# Autodesk Inventor assembly: КВ33.000.100 - Блок переключение передач
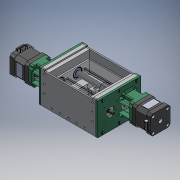
[picture p0: Inventor's stored thumbnail of the model, 180x180]
Saved by Autodesk Inventor 2019 (Build 230136000, 136)
## iProperties
Created: 2021-02-22
Part Number: КВ33.000.100 - Блок переключение передач
Material: Типовые
Document SubType Name: Assembly
Designer: Петров Иван
Author: Петров Иван
## Documents named in this file (13)
- E:\IVAN\Ivan_desktop\Kvantorium\Projects\tractor\design\КВ33.000.100 - Блок переключение передач.iam
- E:\IVAN\Ivan_desktop\Kvantorium\Projects\tractor\design\КВ33.000.101 - Площадка крепежная.ipt
- E:\IVAN\Ivan_desktop\Kvantorium\Projects\tractor\design\design_models\крышка КП.ipt
- E:\IVAN\Ivan_desktop\Kvantorium\Projects\tractor\design\КВ33.000.102 - Стенка толстая.ipt
- E:\IVAN\Ivan_desktop\Kvantorium\Projects\tractor\design\standart_components\Подшипник 626Z.ipt
- E:\IVAN\Ivan_desktop\Kvantorium\Projects\tractor\design\КВ33.000.103 - Стенка тонкая.ipt
- C:\Users\Петров Иван\Documents\Inventor\Content Center Files\R2019\en-US\AS 1427(03)\AS 1427 - M3,5 x 10(1).ipt
- E:\IVAN\Ivan_desktop\Kvantorium\Projects\tractor\design\КВ33.000.104 - Вал.ipt
- E:\IVAN\Ivan_desktop\Kvantorium\Projects\tractor\design\КВ33.000.105 - Каретка.ipt
- E:\IVAN\Ivan_desktop\Kvantorium\Projects\tractor\design\КВ33.000.106 - Муфта.ipt
- E:\IVAN\Ivan_desktop\Kvantorium\Projects\tractor\design\КВ33.000.107 - Крепеж мотора.ipt
- E:\IVAN\Ivan_desktop\Kvantorium\Projects\tractor\design\standart_components\nema 17 motor.ipt
- E:\IVAN\Ivan_desktop\Kvantorium\Projects\tractor\design\for manufacturing\step\КВ33.000.108 - Заслонка.ipt
## Components (43 placed, 12 different names)
1. крышка КП:1 — Flush:1, Mate:1, Mate:2
2. КВ33.000.101 - Площадка крепежная:1 — Flush:1, Mate:1, Mate:2, Mate:3, Flush:2, Mate:4, Mate:5, Flush:3, Mate:6
3. КВ33.000.102 - Стенка толстая:1 — Mate:5, Flush:3, Mate:6, Insert:3, Insert:4, Mate:13, Mate:14, Mate:15, Mate:16, Mate:17, Mate:23, Mate:26, Mate:27, Mate:29, Flush:5, Mate:32, Mate:37, Flush:6, Mate:58, Mate:61
4. КВ33.000.102 - Стенка толстая:2 — Mate:3, Flush:2, Mate:4, Insert:1, Insert:2, Flush:4, Mate:18, Mate:19, Mate:20, Mate:21, Mate:22, Mate:24, Mate:25, Mate:36, Flush:7, Mate:40, Mate:59, Mate:60
5. Подшипник 626Z:1 — Insert:1
6. Подшипник 626Z:2 — Insert:2
7. Подшипник 626Z:3 — Insert:3, Mate:28
8. Подшипник 626Z:4 — Insert:4
9. КВ33.000.103 - Стенка тонкая:1 — Flush:4, Mate:24, Mate:25, Mate:26
10. КВ33.000.103 - Стенка тонкая:2 — Mate:23, Mate:57
11. КВ33.000.104 - Вал:1 — Mate:27, Mate:28, Mate:30, Mate:55
12. КВ33.000.104 - Вал:2 — Mate:29, Flush:5, Mate:31, Mate:34, Mate:56
13. КВ33.000.105 - Каретка:1 — Mate:30, Tangent:1, Mate:60
14. КВ33.000.105 - Каретка:2 — Mate:31, Mate:61, Tangent:2
15. КВ33.000.106 - Муфта:1 — Mate:32, Mate:38, Mate:55
16. КВ33.000.106 - Муфта:2 — Mate:34, Mate:36, Mate:39, Mate:56
17. КВ33.000.107 - Крепеж мотора:1 — Mate:39, Flush:7, Mate:40, Mate:41, Flush:8, Flush:9, Mate:49, Mate:50, Mate:51, Mate:52, Mate:53, Mate:54
18. КВ33.000.107 - Крепеж мотора:2 — Mate:37, Mate:38, Flush:6, Flush:10, Flush:11, Mate:42, Mate:43, Mate:44, Mate:45, Mate:46, Mate:47, Mate:48
19. nema 17 motor:1 — Mate:41, Flush:8, Flush:9
20. nema 17 motor:2 — Flush:10, Flush:11, Mate:42
21. КВ33.000.108 - Заслонка:1 — Mate:57, Mate:58, Mate:59, Tangent:1, Tangent:2
22. AS 1427 - Metric M3,5 x 10:11 — Mate:43
23. AS 1427 - Metric M3,5 x 10:12 — Mate:44
24. AS 1427 - Metric M3,5 x 10:13 — Mate:45
25. AS 1427 - Metric M3,5 x 10:14 — Mate:46
26. AS 1427 - Metric M3,5 x 10:15 — Mate:47
27. AS 1427 - Metric M3,5 x 10:16 — Mate:48
28. AS 1427 - Metric M3,5 x 10:17 — Mate:49
29. AS 1427 - Metric M3,5 x 10:18 — Mate:50
30. AS 1427 - Metric M3,5 x 10:19 — Mate:51
31. AS 1427 - Metric M3,5 x 10:20 — Mate:52
32. AS 1427 - Metric M3,5 x 10:21 — Mate:53
33. AS 1427 - Metric M3,5 x 10:22 — Mate:54
34. AS 1427 - Metric M3,5 x 10:1 — Mate:13
35. AS 1427 - Metric M3,5 x 10:2 — Mate:14
36. AS 1427 - Metric M3,5 x 10:3 — Mate:15
37. AS 1427 - Metric M3,5 x 10:4 — Mate:16
38. AS 1427 - Metric M3,5 x 10:5 — Mate:17
39. AS 1427 - Metric M3,5 x 10:6 — Mate:18
40. AS 1427 - Metric M3,5 x 10:7 — Mate:19
41. AS 1427 - Metric M3,5 x 10:8 — Mate:20
42. AS 1427 - Metric M3,5 x 10:9 — Mate:21
43. AS 1427 - Metric M3,5 x 10:10 — Mate:22
## Relationships (70: Mate 53, Flush 11, Insert 4, Tangent 2)
- Flush:1 (-15 mm): крышка КП:1 ↔ КВ33.000.101 - Площадка крепежная:1
- Mate:1: крышка КП:1 ↔ КВ33.000.101 - Площадка крепежная:1
- Mate:2: крышка КП:1 ↔ КВ33.000.101 - Площадка крепежная:1
- Mate:3: КВ33.000.101 - Площадка крепежная:1 ↔ КВ33.000.102 - Стенка толстая:2
- Flush:2: КВ33.000.101 - Площадка крепежная:1 ↔ КВ33.000.102 - Стенка толстая:2
- Mate:4: КВ33.000.101 - Площадка крепежная:1 ↔ КВ33.000.102 - Стенка толстая:2
- Mate:5: КВ33.000.101 - Площадка крепежная:1 ↔ КВ33.000.102 - Стенка толстая:1
- Flush:3: КВ33.000.101 - Площадка крепежная:1 ↔ КВ33.000.102 - Стенка толстая:1
- Mate:6: КВ33.000.101 - Площадка крепежная:1 ↔ КВ33.000.102 - Стенка толстая:1
- Insert:1: КВ33.000.102 - Стенка толстая:2 ↔ Подшипник 626Z:1
- Insert:2: КВ33.000.102 - Стенка толстая:2 ↔ Подшипник 626Z:2
- Insert:3: КВ33.000.102 - Стенка толстая:1 ↔ Подшипник 626Z:3
- Insert:4: КВ33.000.102 - Стенка толстая:1 ↔ Подшипник 626Z:4
- Flush:4: КВ33.000.102 - Стенка толстая:2 ↔ КВ33.000.103 - Стенка тонкая:1
- Mate:13: КВ33.000.102 - Стенка толстая:1 ↔ AS 1427 - Metric M3,5 x 10:1
- Mate:14: КВ33.000.102 - Стенка толстая:1 ↔ AS 1427 - Metric M3,5 x 10:2
- Mate:15: КВ33.000.102 - Стенка толстая:1 ↔ AS 1427 - Metric M3,5 x 10:3
- Mate:16: КВ33.000.102 - Стенка толстая:1 ↔ AS 1427 - Metric M3,5 x 10:4
- Mate:17: КВ33.000.102 - Стенка толстая:1 ↔ AS 1427 - Metric M3,5 x 10:5
- Mate:18: КВ33.000.102 - Стенка толстая:2 ↔ AS 1427 - Metric M3,5 x 10:6
- Mate:19: КВ33.000.102 - Стенка толстая:2 ↔ AS 1427 - Metric M3,5 x 10:7
- Mate:20: КВ33.000.102 - Стенка толстая:2 ↔ AS 1427 - Metric M3,5 x 10:8
- Mate:21: КВ33.000.102 - Стенка толстая:2 ↔ AS 1427 - Metric M3,5 x 10:9
- Mate:22: КВ33.000.102 - Стенка толстая:2 ↔ AS 1427 - Metric M3,5 x 10:10
- Mate:23: КВ33.000.102 - Стенка толстая:1 ↔ КВ33.000.103 - Стенка тонкая:2
- Mate:24: КВ33.000.102 - Стенка толстая:2 ↔ КВ33.000.103 - Стенка тонкая:1
- Mate:25: КВ33.000.102 - Стенка толстая:2 ↔ КВ33.000.103 - Стенка тонкая:1
- Mate:26: КВ33.000.102 - Стенка толстая:1 ↔ КВ33.000.103 - Стенка тонкая:1
- Mate:27: КВ33.000.102 - Стенка толстая:1 ↔ КВ33.000.104 - Вал:1
- Mate:28: Подшипник 626Z:3 ↔ КВ33.000.104 - Вал:1
- Mate:29: КВ33.000.102 - Стенка толстая:1 ↔ КВ33.000.104 - Вал:2
- Flush:5: КВ33.000.102 - Стенка толстая:1 ↔ КВ33.000.104 - Вал:2
- Mate:30: КВ33.000.104 - Вал:1 ↔ КВ33.000.105 - Каретка:1
- Mate:31: КВ33.000.104 - Вал:2 ↔ КВ33.000.105 - Каретка:2
- Mate:32: КВ33.000.102 - Стенка толстая:1 ↔ КВ33.000.106 - Муфта:1
- Mate:34: КВ33.000.104 - Вал:2 ↔ КВ33.000.106 - Муфта:2
- Mate:36 (3 mm): КВ33.000.102 - Стенка толстая:2 ↔ КВ33.000.106 - Муфта:2
- Mate:37: КВ33.000.102 - Стенка толстая:1 ↔ КВ33.000.107 - Крепеж мотора:2
- Mate:38: КВ33.000.106 - Муфта:1 ↔ КВ33.000.107 - Крепеж мотора:2
- Flush:6: КВ33.000.102 - Стенка толстая:1 ↔ КВ33.000.107 - Крепеж мотора:2
- Mate:39: КВ33.000.106 - Муфта:2 ↔ КВ33.000.107 - Крепеж мотора:1
- Flush:7: КВ33.000.102 - Стенка толстая:2 ↔ КВ33.000.107 - Крепеж мотора:1
- Mate:40: КВ33.000.102 - Стенка толстая:2 ↔ КВ33.000.107 - Крепеж мотора:1
- Mate:41: КВ33.000.107 - Крепеж мотора:1 ↔ nema 17 motor:1
- Flush:8: КВ33.000.107 - Крепеж мотора:1 ↔ nema 17 motor:1
- Flush:9: КВ33.000.107 - Крепеж мотора:1 ↔ nema 17 motor:1
- Flush:10: КВ33.000.107 - Крепеж мотора:2 ↔ nema 17 motor:2
- Flush:11: КВ33.000.107 - Крепеж мотора:2 ↔ nema 17 motor:2
- Mate:42: КВ33.000.107 - Крепеж мотора:2 ↔ nema 17 motor:2
- Mate:43: КВ33.000.107 - Крепеж мотора:2 ↔ AS 1427 - Metric M3,5 x 10:11
- Mate:44: КВ33.000.107 - Крепеж мотора:2 ↔ AS 1427 - Metric M3,5 x 10:12
- Mate:45: КВ33.000.107 - Крепеж мотора:2 ↔ AS 1427 - Metric M3,5 x 10:13
- Mate:46: КВ33.000.107 - Крепеж мотора:2 ↔ AS 1427 - Metric M3,5 x 10:14
- Mate:47: КВ33.000.107 - Крепеж мотора:2 ↔ AS 1427 - Metric M3,5 x 10:15
- Mate:48: КВ33.000.107 - Крепеж мотора:2 ↔ AS 1427 - Metric M3,5 x 10:16
- Mate:49: КВ33.000.107 - Крепеж мотора:1 ↔ AS 1427 - Metric M3,5 x 10:17
- Mate:50: КВ33.000.107 - Крепеж мотора:1 ↔ AS 1427 - Metric M3,5 x 10:18
- Mate:51: КВ33.000.107 - Крепеж мотора:1 ↔ AS 1427 - Metric M3,5 x 10:19
- Mate:52: КВ33.000.107 - Крепеж мотора:1 ↔ AS 1427 - Metric M3,5 x 10:20
- Mate:53: КВ33.000.107 - Крепеж мотора:1 ↔ AS 1427 - Metric M3,5 x 10:21
- Mate:54: КВ33.000.107 - Крепеж мотора:1 ↔ AS 1427 - Metric M3,5 x 10:22
- Mate:55: КВ33.000.104 - Вал:1 ↔ КВ33.000.106 - Муфта:1
- Mate:56: КВ33.000.104 - Вал:2 ↔ КВ33.000.106 - Муфта:2
- Mate:57: КВ33.000.103 - Стенка тонкая:2 ↔ КВ33.000.108 - Заслонка:1
- Mate:58: КВ33.000.102 - Стенка толстая:1 ↔ КВ33.000.108 - Заслонка:1
- Mate:59: КВ33.000.102 - Стенка толстая:2 ↔ КВ33.000.108 - Заслонка:1
- Tangent:1: КВ33.000.105 - Каретка:1 ↔ КВ33.000.108 - Заслонка:1
- Mate:60: КВ33.000.102 - Стенка толстая:2 ↔ КВ33.000.105 - Каретка:1
- Mate:61: КВ33.000.102 - Стенка толстая:1 ↔ КВ33.000.105 - Каретка:2
- Tangent:2: КВ33.000.105 - Каретка:2 ↔ КВ33.000.108 - Заслонка:1
